# Autodesk Inventor assembly: wheel_base
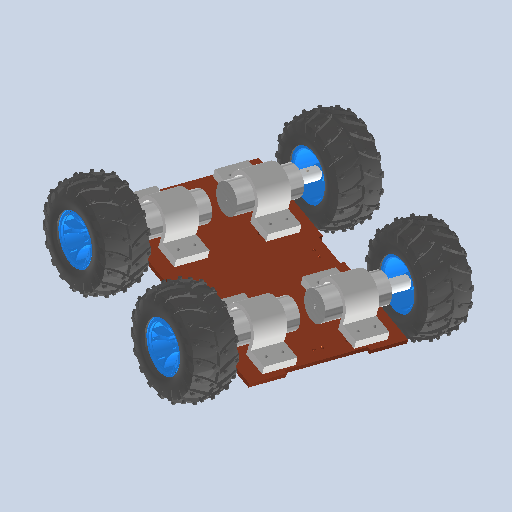
[picture p0: Inventor's stored thumbnail of the model, 512x512]
Saved by Autodesk Inventor 2025.3 (Build 293356030, 356C)
## iProperties
Created: 2026-06-28
Part Number: wheel_base
Document SubType Name: Assembly
Designer: user
Author: user
## Documents named in this file (4)
- C:\Docs\shcool\dojo\Design_3\motor_wheel\wheel_base.iam
- C:\Docs\shcool\dojo\Design_3\chassis_boards\U-bracket.ipt
- C:\Docs\shcool\dojo\Design_3\chassis_boards\base_2.ipt
- C:\Docs\shcool\dojo\Design_3\motor_wheel\motor_wheel_1.iam
## Components (9 placed, 3 different names)
1. U-bracket:1 — Mate:1, Mate:2, Mate:3, Insert:3
2. base_2:1 — Mate:1, Mate:2, Mate:3, Mate:4, Mate:5, Mate:6, Mate:7, Mate:8, Mate:9, Mate:10, Mate:11, Mate:12
3. U-bracket:2 — Mate:7, Mate:11, Mate:12, Insert:2
4. U-bracket:3 — Mate:8, Mate:9, Mate:10, Insert:1
5. U-bracket:4 — Mate:4, Mate:5, Mate:6, Insert:4
6. motor_wheel_1:1 [sub-assembly] — Insert:1
7. motor_wheel_1:2 [sub-assembly] — Insert:2
8. motor_wheel_1:3 [sub-assembly] — Insert:3
9. motor_wheel_1:4 [sub-assembly] — Insert:4
## Relationships (16: Mate 12, Insert 4)
- Mate:1: U-bracket:1 ↔ base_2:1
- Mate:2: U-bracket:1 ↔ base_2:1
- Mate:3: U-bracket:1 ↔ base_2:1
- Mate:4: base_2:1 ↔ U-bracket:4
- Mate:5: base_2:1 ↔ U-bracket:4
- Mate:6: base_2:1 ↔ U-bracket:4
- Mate:7: base_2:1 ↔ U-bracket:2
- Mate:8: base_2:1 ↔ U-bracket:3
- Mate:9: base_2:1 ↔ U-bracket:3
- Mate:10: base_2:1 ↔ U-bracket:3
- Mate:11: base_2:1 ↔ U-bracket:2
- Mate:12: base_2:1 ↔ U-bracket:2
- Insert:1 (-20 mm): U-bracket:3 ↔ motor_wheel_1:1
- Insert:2 (-20 mm): U-bracket:2 ↔ motor_wheel_1:2
- Insert:3 (-20 mm): U-bracket:1 ↔ motor_wheel_1:3
- Insert:4 (20 mm): U-bracket:4 ↔ motor_wheel_1:4
